# Autodesk Inventor assembly: Assembly4
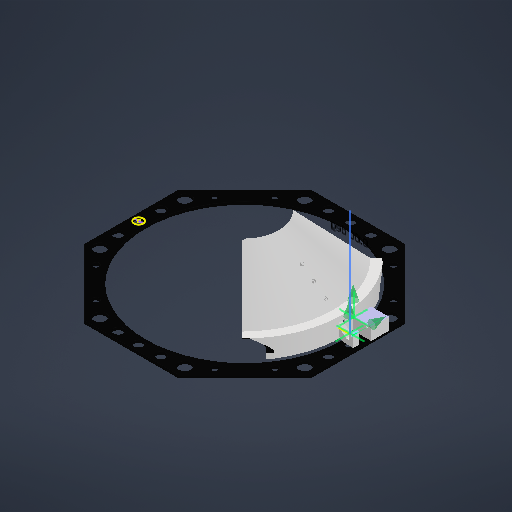
[picture p0: Inventor's stored thumbnail of the model, 512x512]
Saved by Autodesk Inventor 2026.2 (Build 302298000, 298)
## iProperties
Created: 2025-12-16
Part Number: Assembly4
Document SubType Name: Assembly
Designer: Thoma
Author: Thoma
## Documents named in this file (6)
- C:\Users\Thoma\OneDrive\Desktop\Inventor\Quarter_Open\Version_2_Cone\Assembly4.iam
- C:\Users\Thoma\OneDrive\Desktop\Inventor\Quarter_Open\Version_2_Cone\rod_v2.ipt
- C:\Users\Thoma\OneDrive\Desktop\Inventor\Quarter_Open\Version_2_Cone\Telescope_End.ipt
- C:\Users\Thoma\OneDrive\Desktop\Inventor\Quarter_Open\Version_2_Cone\bruh2.ipt
- C:\Users\Thoma\OneDrive\Desktop\Inventor\Quarter_Open\Version_2_Cone\Cover_Lower_Hole.ipt
- C:\Users\Thoma\OneDrive\Desktop\Inventor\Quarter_Open\Version_2_Cone\4mm_0.5_Screw.ipt
## Components (5 placed, 5 different names)
1. Telescope_End:1 — Mate:1, Angle:2, Mate:2
2. bruh2:1 — Mate:1, Angle:2, Mate:2, Mate:3, Mate:4, Angle:3
3. rod_v2:1 — Mate:3, Mate:4, Mate:5, Mate:6, Mate:8, Angle:3, Mate:9
4. Cover_Lower_Hole:1 — Mate:5, Mate:6, Flush:1, Mate:9
5. 4mm_0.5_Screw:1 — Mate:8, Flush:1
## Relationships (11: Mate 8, Angle 2, Flush 1)
- Mate:1: Telescope_End:1 ↔ bruh2:1
- Angle:2 (0 deg): Telescope_End:1 ↔ bruh2:1
- Mate:2: Telescope_End:1 ↔ bruh2:1
- Mate:3: bruh2:1 ↔ rod_v2:1
- Mate:4 (15.55 mm): bruh2:1 ↔ rod_v2:1
- Mate:5: rod_v2:1 ↔ Cover_Lower_Hole:1
- Mate:6: rod_v2:1 ↔ Cover_Lower_Hole:1
- Mate:8: rod_v2:1 ↔ 4mm_0.5_Screw:1
- Flush:1 (-5 mm): Cover_Lower_Hole:1 ↔ 4mm_0.5_Screw:1
- Angle:3 (0 deg): bruh2:1 ↔ rod_v2:1
- Mate:9 (-12 mm): rod_v2:1 ↔ Cover_Lower_Hole:1
